# Autodesk Inventor assembly: E000-Compresseur
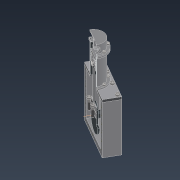
[picture p0: Inventor's stored thumbnail of the model, 180x180]
Saved by Autodesk Inventor 2021.3 (Build 253353000, 353)
## iProperties
Created: 2022-03-31
Part Number: E000-Compresseur
Document SubType Name: Assembly
Designer: remi
Author: remi
## Documents named in this file (8)
- C:\Users\remi\OneDrive\Documents\Cours\05-HEVS\S2fb\mechanic\CCo\project\Compressor\E000-Compresseur.iam
- C:\Users\remi\OneDrive\Documents\Cours\05-HEVS\S2fb\mechanic\CCo\project\Compressor\E001-Chambre.iam
- C:\Users\remi\OneDrive\Documents\Cours\05-HEVS\S2fb\mechanic\CCo\project\Compressor\E002-Piston.iam
- C:\Users\remi\OneDrive\Documents\Cours\05-HEVS\S2fb\mechanic\CCo\project\Compressor\E005-Bielle.iam
- C:\Users\remi\OneDrive\Documents\Cours\05-HEVS\S2fb\mechanic\CCo\project\Compressor\R2021\en-US\Bearing GB_T 5800-2003\Rolling bearing GB_T 5800-2003 -639_3.ipt
- C:\Users\remi\OneDrive\Documents\Cours\05-HEVS\S2fb\mechanic\CCo\project\Compressor\E006-Carter.iam
- C:\Users\remi\OneDrive\Documents\Cours\05-HEVS\S2fb\mechanic\CCo\project\Compressor\R2021\en-US\AS 1420\AS 1420 - 1973 - M3 x 8.ipt
- C:\Users\remi\OneDrive\Documents\Cours\05-HEVS\S2fb\mechanic\CCo\project\Compressor\R2021\en-US\AS 1420\AS 1420 - 1973 - M4 x 12.ipt
## Components (19 placed, 7 different names)
1. E001-Chambre:1 [sub-assembly] — Mate:1, Mate:5, Mate:7, Mate:8, Insert:1, Insert:2, Insert:3, Insert:4, Insert:5, Insert:6
2. E002-Piston:1 [sub-assembly] — Mate:1, Mate:2, Mate:3
3. E005-Bielle:1 [sub-assembly] — Mate:2, Mate:4
4. Bearing GB/T 5800-2003 639/3:1 — Mate:3
5. E006-Carter:1 [sub-assembly] — Mate:4, Mate:5, Mate:7, Mate:8, Mate:9, Angle:1, Insert:7, Insert:8, Insert:9, Insert:10, Insert:11, Insert:12, Insert:13, Insert:14
6. AS 1420 - Metric M3 x 8:1 — Insert:1
7. AS 1420 - Metric M3 x 8:2 — Insert:2
8. AS 1420 - Metric M3 x 8:3 — Insert:3
9. AS 1420 - Metric M3 x 8:4 — Insert:4
10. AS 1420 - Metric M3 x 8:5 — Insert:5
11. AS 1420 - Metric M3 x 8:6 — Insert:6
12. AS 1420 - Metric M4 x 12:1 — Insert:7
13. AS 1420 - Metric M4 x 12:2 — Insert:8
14. AS 1420 - Metric M4 x 12:3 — Insert:9
15. AS 1420 - Metric M4 x 12:4 — Insert:10
16. AS 1420 - Metric M4 x 12:5 — Insert:11
17. AS 1420 - Metric M4 x 12:6 — Insert:12
18. AS 1420 - Metric M4 x 12:7 — Insert:13
19. AS 1420 - Metric M4 x 12:8 — Insert:14
## Relationships (23: Insert 14, Mate 8, Angle 1)
- Mate:1: E001-Chambre:1 ↔ E002-Piston:1
- Mate:2: E002-Piston:1 ↔ E005-Bielle:1
- Mate:3: E002-Piston:1 ↔ Bearing GB/T 5800-2003 639/3:1
- Mate:4: E005-Bielle:1 ↔ E006-Carter:1
- Mate:5: E001-Chambre:1 ↔ E006-Carter:1
- Mate:7: E001-Chambre:1 ↔ E006-Carter:1
- Mate:8: E001-Chambre:1 ↔ E006-Carter:1
- Insert:1: E001-Chambre:1 ↔ AS 1420 - Metric M3 x 8:1
- Insert:2: E001-Chambre:1 ↔ AS 1420 - Metric M3 x 8:2
- Insert:3: E001-Chambre:1 ↔ AS 1420 - Metric M3 x 8:3
- Insert:4: E001-Chambre:1 ↔ AS 1420 - Metric M3 x 8:4
- Insert:5: E001-Chambre:1 ↔ AS 1420 - Metric M3 x 8:5
- Insert:6: E001-Chambre:1 ↔ AS 1420 - Metric M3 x 8:6
- Mate:9: E006-Carter:1
- Angle:1 (0 deg): E006-Carter:1
- Insert:7: E006-Carter:1 ↔ AS 1420 - Metric M4 x 12:1
- Insert:8: E006-Carter:1 ↔ AS 1420 - Metric M4 x 12:2
- Insert:9: E006-Carter:1 ↔ AS 1420 - Metric M4 x 12:3
- Insert:10: E006-Carter:1 ↔ AS 1420 - Metric M4 x 12:4
- Insert:11: E006-Carter:1 ↔ AS 1420 - Metric M4 x 12:5
- Insert:12: E006-Carter:1 ↔ AS 1420 - Metric M4 x 12:6
- Insert:13: E006-Carter:1 ↔ AS 1420 - Metric M4 x 12:7
- Insert:14: E006-Carter:1 ↔ AS 1420 - Metric M4 x 12:8
